# Autodesk Inventor assembly: Assembly
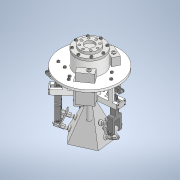
[picture p0: Inventor's stored thumbnail of the model, 180x180]
Saved by Autodesk Inventor 2021 (Build 250183000, 183)
## iProperties
Created: 2020-11-29
Part Number: Assembly
Document SubType Name: Assembly
Designer: awitc
Author: awitc
## Documents named in this file (36)
- C:\Users\awitc\Documents\Mechatronic Engineering\III rok\IndustrialRobots\GripperProject\Assembly.iam
- C:\Users\awitc\Documents\Mechatronic Engineering\III rok\IndustrialRobots\GripperProject\cup.ipt
- C:\Users\awitc\Documents\Mechatronic Engineering\III rok\IndustrialRobots\GripperProject\link.ipt
- C:\Users\awitc\Documents\Mechatronic Engineering\III rok\IndustrialRobots\GripperProject\finger.ipt
- C:\Users\awitc\Documents\Mechatronic Engineering\III rok\IndustrialRobots\GripperProject\actuatorLink.ipt
- C:\Users\awitc\Documents\Mechatronic Engineering\III rok\IndustrialRobots\GripperProject\bracket.ipt
- C:\Users\awitc\Documents\Mechatronic Engineering\III rok\IndustrialRobots\GripperProject\linkToActuator2.ipt
- C:\Users\awitc\Documents\Mechatronic Engineering\III rok\IndustrialRobots\GripperProject\linkToActuator3.ipt
- C:\Users\awitc\Documents\Mechatronic Engineering\III rok\IndustrialRobots\GripperProject\linkToActuator5.ipt
- C:\Users\awitc\Documents\Mechatronic Engineering\III rok\IndustrialRobots\GripperProject\linkToActuator4.ipt
- C:\Users\awitc\Documents\Mechatronic Engineering\III rok\IndustrialRobots\GripperProject\joint.ipt
- C:\Users\awitc\Documents\Mechatronic Engineering\III rok\IndustrialRobots\GripperProject\pneumaticActuator.ipt
- C:\Users\awitc\Documents\Mechatronic Engineering\III rok\IndustrialRobots\GripperProject\actuatorMountingPlate.ipt
- C:\Users\awitc\Documents\Mechatronic Engineering\III rok\IndustrialRobots\GripperProject\spacer.ipt
- C:\Users\awitc\Documents\Mechatronic Engineering\III rok\IndustrialRobots\GripperProject\vacuumGenerator.ipt
- C:\Users\awitc\Documents\Mechatronic Engineering\III rok\IndustrialRobots\GripperProject\mountingPlate.ipt
- C:\Users\awitc\Documents\Mechatronic Engineering\III rok\IndustrialRobots\GripperProject\pipeJoint.ipt
- C:\Users\awitc\Documents\Mechatronic Engineering\III rok\IndustrialRobots\GripperProject\customPin.ipt
- C:\Users\awitc\Documents\Inventor\Content Center Files\R2021\en-US\DIN 84\DIN 84 - M3 x 8.ipt
- C:\Users\awitc\Documents\Inventor\Content Center Files\R2021\en-US\DIN 84\DIN 84 - M1 x 8.ipt
- C:\Users\awitc\Documents\Inventor\Content Center Files\R2021\en-US\DIN 84\DIN 84 - M3 x 28.ipt
- C:\Users\awitc\Documents\Inventor\Content Center Files\R2021\en-US\DIN 439-2\DIN 439 - M3 x 0,5.ipt
- C:\Users\awitc\Documents\Inventor\Content Center Files\R2021\en-US\DIN 84\DIN 84 - M3 x 6.ipt
- C:\Users\awitc\Documents\Inventor\Content Center Files\R2021\en-US\DIN 125-1  A\DIN 125 - A 3,2.ipt
- C:\Users\awitc\Documents\Inventor\Content Center Files\R2021\en-US\DIN 84\DIN 84 - M3 x 14.ipt
- C:\Users\awitc\Documents\Mechatronic Engineering\III rok\IndustrialRobots\GripperProject\holder.ipt
- C:\Users\awitc\Documents\Inventor\Content Center Files\R2021\en-US\DIN 84\DIN 84 - M3 x 12.ipt
- C:\Users\awitc\Documents\Inventor\Content Center Files\R2021\en-US\DIN 84\DIN 84 - M3 x 25.ipt
- C:\Users\awitc\Documents\Mechatronic Engineering\III rok\IndustrialRobots\GripperProject\upperBasePart1.ipt
- C:\Users\awitc\Documents\Mechatronic Engineering\III rok\IndustrialRobots\GripperProject\upperBasePart2.ipt
- C:\Users\awitc\Documents\Mechatronic Engineering\III rok\IndustrialRobots\GripperProject\basePart1.ipt
- C:\Users\awitc\Documents\Mechatronic Engineering\III rok\IndustrialRobots\GripperProject\basePart2.ipt
- C:\Users\awitc\Documents\Mechatronic Engineering\III rok\IndustrialRobots\GripperProject\WK330.ipt
- C:\Users\awitc\Documents\Mechatronic Engineering\III rok\IndustrialRobots\GripperProject\sensorMount.ipt
- C:\Users\awitc\Documents\Mechatronic Engineering\III rok\IndustrialRobots\GripperProject\largePart.ipt
- C:\Users\awitc\Documents\Mechatronic Engineering\III rok\IndustrialRobots\GripperProject\Part4.ipt
## Components (142 placed, 35 different names)
1. bracket:1 — Insert:297, Insert:298, Insert:299, Insert:300, Insert:391, Insert:392
2. bracket:2 — Insert:301, Insert:302, Insert:303, Insert:304, Insert:395, Insert:396
3. bracket:3 — Insert:305, Insert:306, Insert:307, Insert:308, Insert:393, Insert:394
4. link:7 — Insert:144, Insert:145, Insert:169, Insert:174, Rigid:1, Insert:411, Insert:412, Mate:61, Flush:14
5. cup:14 — Insert:144
6. cup:16 — Insert:145, Insert:412
7. joint:1 — Insert:175, Rigid:1
8. pneumaticActuator:1 — Insert:159, Insert:160, Cylindrical:1
9. actuatorMountingPlate:1 — Insert:159, Insert:160, Insert:163, Insert:164, Insert:390, Flush:8
10. spacer:1 — Insert:163, Insert:164, Mate:59, Insert:410
11. vacuumGenerator:2 — Mate:36, Mate:37, Flush:1
12. mountingPlate:1 — Insert:339, Insert:340, Insert:341, Insert:342, Insert:343, Insert:344, Insert:345, Insert:346, Mate:58, Insert:409
13. pipeJoint:1 — Insert:169
14. pipeJoint:6 — Insert:174, Insert:411
15. finger:1 — Insert:175, Insert:255, Insert:294, Insert:311, Insert:312, Insert:324, Flush:9
16. link:8 — Insert:413, Insert:414
17. cup:17
18. cup:18 — Insert:413
19. joint:2 — Insert:189
20. pipeJoint:7
21. pipeJoint:8 — Insert:414
22. finger:2 — Insert:189, Insert:243, Insert:295, Insert:310, Insert:313, Insert:325, Flush:11
23. link:9 — Insert:415, Insert:416
24. cup:19
25. cup:20 — Insert:415
26. joint:3
27. pipeJoint:9
28. pipeJoint:10 — Insert:416
29. finger:3 — Insert:266, Insert:296, Insert:309, Insert:314, Insert:323, Flush:10
30. linkToActuator2:1 — Insert:244, Insert:245, Insert:292, Insert:293, Insert:397
31. linkToActuator3:1 — Insert:246, Insert:247, Insert:286, Insert:291, Insert:398
32. linkToActuator4:1 — Insert:245, Insert:246
33. linkToActuator5:1 — Insert:243, Insert:244
34. actuatorLink:1 — Insert:273, Cylindrical:1, Insert:274, Insert:275, Insert:315, Insert:316, Insert:317, Insert:318, Insert:319, Insert:320
35. linkToActuator5:2 — Insert:247, Insert:275
36. linkToActuator2:2 — Insert:288, Insert:289, Insert:401
37. linkToActuator3:2 — Insert:287, Insert:290, Insert:402
38. linkToActuator4:2
39. linkToActuator5:3 — Insert:255
40. linkToActuator5:4 — Insert:273
41. linkToActuator2:3 — Insert:265, Insert:282, Insert:284, Insert:399
42. linkToActuator3:3 — Insert:283, Insert:285, Insert:400
43. linkToActuator4:3
44. linkToActuator5:6 — Insert:274
45. linkToActuator5:7 — Insert:265, Insert:266
46. customPin:1 — Insert:282
47. customPin:2 — Insert:283
48. customPin:3 — Insert:285
49. customPin:4 — Insert:287
50. customPin:5 — Insert:286
51. customPin:6 — Insert:284
52. customPin:7 — Insert:288
53. customPin:8 — Insert:289
54. customPin:9 — Insert:290
55. customPin:10 — Insert:291
56. customPin:11 — Insert:292
57. customPin:12 — Insert:293
58. DIN 84 - replaced by DIN EN ISO 1207 M1 x 8:1 — Insert:299
59. DIN 84 - replaced by DIN EN ISO 1207 M1 x 8:2 — Insert:298
60. DIN 84 - replaced by DIN EN ISO 1207 M1 x 8:3 — Insert:297
61. DIN 84 - replaced by DIN EN ISO 1207 M1 x 8:4 — Insert:300
62. DIN 84 - replaced by DIN EN ISO 1207 M3 x 28:1 — Insert:296
63. DIN 84 - replaced by DIN EN ISO 1207 M3 x 28:2 — Insert:295
64. DIN 84 - replaced by DIN EN ISO 1207 M3 x 28:3 — Insert:294
65. DIN 84 - replaced by DIN EN ISO 1207 M1 x 8:5 — Insert:302
66. DIN 84 - replaced by DIN EN ISO 1207 M1 x 8:6 — Insert:303
67. DIN 84 - replaced by DIN EN ISO 1207 M1 x 8:7 — Insert:304
68. DIN 84 - replaced by DIN EN ISO 1207 M1 x 8:8 — Insert:301
69. DIN 84 - replaced by DIN EN ISO 1207 M1 x 8:10 — Insert:305
70. DIN 84 - replaced by DIN EN ISO 1207 M1 x 8:9 — Insert:308
71. DIN 84 - replaced by DIN EN ISO 1207 M1 x 8:11 — Insert:307
72. DIN 84 - replaced by DIN EN ISO 1207 M1 x 8:12 — Insert:306
73. DIN 439-2 - replaced by DIN EN 24035/28675 M3:1 — Insert:312
74. DIN 439-2 - replaced by DIN EN 24035/28675 M3:2 — Insert:314
75. DIN 439-2 - replaced by DIN EN 24035/28675 M3:4 — Insert:313
76. DIN 84 - replaced by DIN EN ISO 1207 M3 x 6:1 — Insert:309
77. DIN 84 - replaced by DIN EN ISO 1207 M3 x 6:2 — Insert:310
78. DIN 84 - replaced by DIN EN ISO 1207 M3 x 6:4 — Insert:311
79. DIN 84 - replaced by DIN EN ISO 1207 M3 x 6:5 — Insert:315
80. DIN 439-2 - replaced by DIN EN 24035/28675 M3:5 — Insert:316
81. DIN 439-2 - replaced by DIN EN 24035/28675 M3:6 — Insert:318
82. DIN 84 - replaced by DIN EN ISO 1207 M3 x 6:6 — Insert:317
83. DIN 84 - replaced by DIN EN ISO 1207 M3 x 6:7 — Insert:319
84. DIN 439-2 - replaced by DIN EN 24035/28675 M3:7 — Insert:320
85. DIN 125-1 A A 3,2:1 — Insert:323, Insert:330
86. DIN 125-1 A A 3,2:2 — Insert:336, Insert:407
87. DIN 125-1 A A 3,2:3 — Insert:337, Insert:406
88. DIN 125-1 A A 3,2:4 — Insert:324, Insert:331
89. DIN 125-1 A A 3,2:5 — Insert:325, Insert:332
90. DIN 125-1 A A 3,2:6 — Insert:333, Insert:405
91. DIN 125-1 A A 3,2:7 — Insert:338, Insert:408
92. DIN 125-1 A A 3,2:8 — Insert:334, Insert:404
93. DIN 125-1 A A 3,2:9 — Insert:335, Insert:403
94. DIN 439-2 - replaced by DIN EN 24035/28675 M3:8 — Insert:330
95. DIN 439-2 - replaced by DIN EN 24035/28675 M3:9 — Insert:331
96. DIN 439-2 - replaced by DIN EN 24035/28675 M3:10 — Insert:332
97. DIN 439-2 - replaced by DIN EN 24035/28675 M3:11 — Insert:333
98. DIN 439-2 - replaced by DIN EN 24035/28675 M3:12 — Insert:334
99. DIN 439-2 - replaced by DIN EN 24035/28675 M3:13 — Insert:335
100. DIN 439-2 - replaced by DIN EN 24035/28675 M3:14 — Insert:336
101. DIN 439-2 - replaced by DIN EN 24035/28675 M3:15 — Insert:337
102. DIN 439-2 - replaced by DIN EN 24035/28675 M3:16 — Insert:338
103. DIN 84 - replaced by DIN EN ISO 1207 M3 x 14:1 — Insert:345
104. DIN 84 - replaced by DIN EN ISO 1207 M3 x 14:2 — Insert:344
105. DIN 84 - replaced by DIN EN ISO 1207 M3 x 14:3 — Insert:343
106. DIN 84 - replaced by DIN EN ISO 1207 M3 x 14:4 — Insert:342
107. DIN 84 - replaced by DIN EN ISO 1207 M3 x 14:5 — Insert:341
108. DIN 84 - replaced by DIN EN ISO 1207 M3 x 14:6 — Insert:339
109. DIN 84 - replaced by DIN EN ISO 1207 M3 x 14:7 — Insert:340
110. DIN 84 - replaced by DIN EN ISO 1207 M3 x 14:9 — Insert:346
111. holder:1 — Mate:36, Mate:37, Flush:1, Insert:365, Insert:366, Insert:378, Insert:379
112. DIN 439-2 - replaced by DIN EN 24035/28675 M3:18 — Insert:365
113. DIN 439-2 - replaced by DIN EN 24035/28675 M3:19 — Insert:366
114. basePart1:1 — Mate:47, Flush:4, Mate:48, Mate:49, Flush:5, Mate:50, Mate:51, Flush:6, Insert:390, Mate:57, Flush:8
115. basePart2:1 — Mate:50, Mate:51, Flush:6, Insert:393, Insert:394, Insert:399, Insert:400, Flush:10, Insert:405, Insert:408
116. basePart2:2 — Mate:47, Flush:4, Mate:57, Insert:391, Insert:392, Insert:401, Insert:402, Flush:9, Insert:406, Insert:407
117. basePart2:3 — Mate:48, Mate:49, Flush:5, Insert:395, Insert:396, Insert:397, Insert:398, Flush:11, Insert:403, Insert:404
118. DIN 84 - replaced by DIN EN ISO 1207 M3 x 12:4 — Insert:381
119. DIN 84 - replaced by DIN EN ISO 1207 M3 x 12:5 — Insert:380
120. DIN 84 - replaced by DIN EN ISO 1207 M3 x 8:1 — Insert:389
121. upperBasePart2:1 — Mate:52, Mate:53, Mate:54, Mate:58, Insert:409
122. upperBasePart1:1 — Insert:369, Insert:370, Insert:371, Insert:372, Insert:373, Mate:52, Mate:53, Mate:54, Insert:376, Insert:377, Insert:378, Insert:379, Insert:380, Insert:381, Insert:382, Insert:383, Insert:384, Insert:385, Insert:386, Insert:387, Insert:388, Insert:389, Mate:59, Insert:410
123. DIN 84 - replaced by DIN EN ISO 1207 M3 x 25:2 — Insert:372
124. DIN 84 - replaced by DIN EN ISO 1207 M3 x 25:3 — Insert:373
125. DIN 84 - replaced by DIN EN ISO 1207 M3 x 25:5 — Insert:371
126. DIN 84 - replaced by DIN EN ISO 1207 M3 x 25:6 — Insert:369
127. DIN 84 - replaced by DIN EN ISO 1207 M3 x 25:7 — Insert:370
128. vacuumGenerator:3
129. holder:2 — Insert:376, Insert:377
130. DIN 439-2 - replaced by DIN EN 24035/28675 M3:20
131. DIN 439-2 - replaced by DIN EN 24035/28675 M3:21
132. DIN 84 - replaced by DIN EN ISO 1207 M3 x 12:6 — Insert:382
133. DIN 84 - replaced by DIN EN ISO 1207 M3 x 12:7 — Insert:383
134. DIN 84 - replaced by DIN EN ISO 1207 M3 x 8:2 — Insert:387
135. DIN 84 - replaced by DIN EN ISO 1207 M3 x 8:4 — Insert:385
136. DIN 84 - replaced by DIN EN ISO 1207 M3 x 8:5 — Insert:386
137. DIN 84 - replaced by DIN EN ISO 1207 M3 x 8:6 — Insert:388
138. DIN 84 - replaced by DIN EN ISO 1207 M3 x 8:7 — Insert:384
139. sensorMount:1 — Flush:12, Mate:60, Flush:13, Mate:61, Flush:14
140. WK330:1 — Flush:12, Mate:60, Flush:13
141. largePart:1 — Mate:62
142. Part4:1 — Mate:62
## Relationships (180: Insert 146, Mate 18, Flush 12, WeldJoint 3, CylindricalJoint 1)
- Insert:144: link:7 ↔ cup:14
- Insert:145: link:7 ↔ cup:16
- Insert:159: pneumaticActuator:1 ↔ actuatorMountingPlate:1
- Insert:160: pneumaticActuator:1 ↔ actuatorMountingPlate:1
- Insert:163: actuatorMountingPlate:1 ↔ spacer:1
- Insert:164: actuatorMountingPlate:1 ↔ spacer:1
- Insert:169: link:7 ↔ pipeJoint:1
- Insert:174: link:7 ↔ pipeJoint:6
- Insert:175: joint:1 ↔ finger:1
- Rigid:1 [WeldJoint]: link:7 ↔ joint:1
- [Insert]: link:8 ↔ cup:17
- [Insert]: link:8 ↔ cup:18
- [Insert]: link:8 ↔ pipeJoint:7
- [Insert]: link:8 ↔ pipeJoint:8
- [WeldJoint]: link:8 ↔ joint:2
- [Insert]: link:9 ↔ cup:19
- [Insert]: link:9 ↔ cup:20
- [Insert]: link:9 ↔ pipeJoint:9
- [Insert]: link:9 ↔ pipeJoint:10
- [Insert]: joint:3 ↔ finger:3
- [WeldJoint]: link:9 ↔ joint:3
- Insert:189: joint:2 ↔ finger:2
- Insert:243: finger:2 ↔ linkToActuator5:1
- Insert:244: linkToActuator2:1 ↔ linkToActuator5:1
- Insert:245: linkToActuator2:1 ↔ linkToActuator4:1
- Insert:246: linkToActuator3:1 ↔ linkToActuator4:1
- Insert:247: linkToActuator3:1 ↔ linkToActuator5:2
- [Insert]: linkToActuator2:2 ↔ linkToActuator5:3
- [Insert]: linkToActuator2:2 ↔ linkToActuator4:2
- [Insert]: linkToActuator3:2 ↔ linkToActuator4:2
- [Insert]: linkToActuator3:2 ↔ linkToActuator5:4
- Insert:255: finger:1 ↔ linkToActuator5:3
- [Insert]: linkToActuator2:3 ↔ linkToActuator4:3
- [Insert]: linkToActuator3:3 ↔ linkToActuator4:3
- [Insert]: linkToActuator3:3 ↔ linkToActuator5:6
- Insert:265: linkToActuator2:3 ↔ linkToActuator5:7
- Insert:266: finger:3 ↔ linkToActuator5:7
- Insert:273: actuatorLink:1 ↔ linkToActuator5:4
- Cylindrical:1: pneumaticActuator:1 ↔ actuatorLink:1
- Insert:274: actuatorLink:1 ↔ linkToActuator5:6
- Insert:275: actuatorLink:1 ↔ linkToActuator5:2
- Insert:282: linkToActuator2:3 ↔ customPin:1
- Insert:283: linkToActuator3:3 ↔ customPin:2
- Insert:284: linkToActuator2:3 ↔ customPin:6
- Insert:285: linkToActuator3:3 ↔ customPin:3
- Insert:286: linkToActuator3:1 ↔ customPin:5
- Insert:287: linkToActuator3:2 ↔ customPin:4
- Insert:288: linkToActuator2:2 ↔ customPin:7
- Insert:289: linkToActuator2:2 ↔ customPin:8
- Insert:290: linkToActuator3:2 ↔ customPin:9
- Insert:291: linkToActuator3:1 ↔ customPin:10
- Insert:292: linkToActuator2:1 ↔ customPin:11
- Insert:293: linkToActuator2:1 ↔ customPin:12
- Insert:294: finger:1 ↔ DIN 84 - replaced by DIN EN ISO 1207 M3 x 28:3
- Insert:295: finger:2 ↔ DIN 84 - replaced by DIN EN ISO 1207 M3 x 28:2
- Insert:296: finger:3 ↔ DIN 84 - replaced by DIN EN ISO 1207 M3 x 28:1
- Insert:297: bracket:1 ↔ DIN 84 - replaced by DIN EN ISO 1207 M1 x 8:3
- Insert:298: bracket:1 ↔ DIN 84 - replaced by DIN EN ISO 1207 M1 x 8:2
- Insert:299: bracket:1 ↔ DIN 84 - replaced by DIN EN ISO 1207 M1 x 8:1
- Insert:300: bracket:1 ↔ DIN 84 - replaced by DIN EN ISO 1207 M1 x 8:4
- Insert:301: bracket:2 ↔ DIN 84 - replaced by DIN EN ISO 1207 M1 x 8:8
- Insert:302: bracket:2 ↔ DIN 84 - replaced by DIN EN ISO 1207 M1 x 8:5
- Insert:303: bracket:2 ↔ DIN 84 - replaced by DIN EN ISO 1207 M1 x 8:6
- Insert:304: bracket:2 ↔ DIN 84 - replaced by DIN EN ISO 1207 M1 x 8:7
- Insert:305: bracket:3 ↔ DIN 84 - replaced by DIN EN ISO 1207 M1 x 8:10
- Insert:306: bracket:3 ↔ DIN 84 - replaced by DIN EN ISO 1207 M1 x 8:12
- Insert:307: bracket:3 ↔ DIN 84 - replaced by DIN EN ISO 1207 M1 x 8:11
- Insert:308: bracket:3 ↔ DIN 84 - replaced by DIN EN ISO 1207 M1 x 8:9
- Insert:309: finger:3 ↔ DIN 84 - replaced by DIN EN ISO 1207 M3 x 6:1
- Insert:310: finger:2 ↔ DIN 84 - replaced by DIN EN ISO 1207 M3 x 6:2
- Insert:311: finger:1 ↔ DIN 84 - replaced by DIN EN ISO 1207 M3 x 6:4
- Insert:312: finger:1 ↔ DIN 439-2 - replaced by DIN EN 24035/28675 M3:1
- Insert:313: finger:2 ↔ DIN 439-2 - replaced by DIN EN 24035/28675 M3:4
- Insert:314: finger:3 ↔ DIN 439-2 - replaced by DIN EN 24035/28675 M3:2
- Insert:315: actuatorLink:1 ↔ DIN 84 - replaced by DIN EN ISO 1207 M3 x 6:5
- Insert:316: actuatorLink:1 ↔ DIN 439-2 - replaced by DIN EN 24035/28675 M3:5
- Insert:317: actuatorLink:1 ↔ DIN 84 - replaced by DIN EN ISO 1207 M3 x 6:6
- Insert:318: actuatorLink:1 ↔ DIN 439-2 - replaced by DIN EN 24035/28675 M3:6
- Insert:319: actuatorLink:1 ↔ DIN 84 - replaced by DIN EN ISO 1207 M3 x 6:7
- Insert:320: actuatorLink:1 ↔ DIN 439-2 - replaced by DIN EN 24035/28675 M3:7
- Insert:323: finger:3 ↔ DIN 125-1 A A 3,2:1
- Insert:324: finger:1 ↔ DIN 125-1 A A 3,2:4
- Insert:325: finger:2 ↔ DIN 125-1 A A 3,2:5
- Insert:330: DIN 125-1 A A 3,2:1 ↔ DIN 439-2 - replaced by DIN EN 24035/28675 M3:8
- Insert:331: DIN 125-1 A A 3,2:4 ↔ DIN 439-2 - replaced by DIN EN 24035/28675 M3:9
- Insert:332: DIN 125-1 A A 3,2:5 ↔ DIN 439-2 - replaced by DIN EN 24035/28675 M3:10
- Insert:333: DIN 125-1 A A 3,2:6 ↔ DIN 439-2 - replaced by DIN EN 24035/28675 M3:11
- Insert:334: DIN 125-1 A A 3,2:8 ↔ DIN 439-2 - replaced by DIN EN 24035/28675 M3:12
- Insert:335: DIN 125-1 A A 3,2:9 ↔ DIN 439-2 - replaced by DIN EN 24035/28675 M3:13
- Insert:336: DIN 125-1 A A 3,2:2 ↔ DIN 439-2 - replaced by DIN EN 24035/28675 M3:14
- Insert:337: DIN 125-1 A A 3,2:3 ↔ DIN 439-2 - replaced by DIN EN 24035/28675 M3:15
- Insert:338: DIN 125-1 A A 3,2:7 ↔ DIN 439-2 - replaced by DIN EN 24035/28675 M3:16
- Insert:339: mountingPlate:1 ↔ DIN 84 - replaced by DIN EN ISO 1207 M3 x 14:6
- Insert:340: mountingPlate:1 ↔ DIN 84 - replaced by DIN EN ISO 1207 M3 x 14:7
- Insert:341: mountingPlate:1 ↔ DIN 84 - replaced by DIN EN ISO 1207 M3 x 14:5
- Insert:342: mountingPlate:1 ↔ DIN 84 - replaced by DIN EN ISO 1207 M3 x 14:4
- Insert:343: mountingPlate:1 ↔ DIN 84 - replaced by DIN EN ISO 1207 M3 x 14:3
- Insert:344: mountingPlate:1 ↔ DIN 84 - replaced by DIN EN ISO 1207 M3 x 14:2
- Insert:345: mountingPlate:1 ↔ DIN 84 - replaced by DIN EN ISO 1207 M3 x 14:1
- Insert:346: mountingPlate:1 ↔ DIN 84 - replaced by DIN EN ISO 1207 M3 x 14:9
- Mate:36: vacuumGenerator:2 ↔ holder:1
- Mate:37: vacuumGenerator:2 ↔ holder:1
- Flush:1: vacuumGenerator:2 ↔ holder:1
- Insert:365: holder:1 ↔ DIN 439-2 - replaced by DIN EN 24035/28675 M3:18
- Insert:366: holder:1 ↔ DIN 439-2 - replaced by DIN EN 24035/28675 M3:19
- Mate:47: basePart1:1 ↔ basePart2:2
- Flush:4: basePart1:1 ↔ basePart2:2
- Mate:48: basePart1:1 ↔ basePart2:3
- Mate:49: basePart1:1 ↔ basePart2:3
- Flush:5: basePart1:1 ↔ basePart2:3
- Mate:50: basePart1:1 ↔ basePart2:1
- Mate:51: basePart1:1 ↔ basePart2:1
- Flush:6: basePart1:1 ↔ basePart2:1
- Insert:369: upperBasePart1:1 ↔ DIN 84 - replaced by DIN EN ISO 1207 M3 x 25:6
- Insert:370: upperBasePart1:1 ↔ DIN 84 - replaced by DIN EN ISO 1207 M3 x 25:7
- Insert:371: upperBasePart1:1 ↔ DIN 84 - replaced by DIN EN ISO 1207 M3 x 25:5
- Insert:372: upperBasePart1:1 ↔ DIN 84 - replaced by DIN EN ISO 1207 M3 x 25:2
- Insert:373: upperBasePart1:1 ↔ DIN 84 - replaced by DIN EN ISO 1207 M3 x 25:3
- Mate:52: upperBasePart2:1 ↔ upperBasePart1:1
- Mate:53: upperBasePart2:1 ↔ upperBasePart1:1
- Mate:54: upperBasePart2:1 ↔ upperBasePart1:1
- [Mate]: vacuumGenerator:3 ↔ holder:2
- [Mate]: vacuumGenerator:3 ↔ holder:2
- [Flush]: vacuumGenerator:3 ↔ holder:2
- [Insert]: holder:2 ↔ DIN 439-2 - replaced by DIN EN 24035/28675 M3:20
- [Insert]: holder:2 ↔ DIN 439-2 - replaced by DIN EN 24035/28675 M3:21
- Insert:376: upperBasePart1:1 ↔ holder:2
- Insert:377: upperBasePart1:1 ↔ holder:2
- Insert:378: holder:1 ↔ upperBasePart1:1
- Insert:379: holder:1 ↔ upperBasePart1:1
- Insert:380: DIN 84 - replaced by DIN EN ISO 1207 M3 x 12:5 ↔ upperBasePart1:1
- Insert:381: DIN 84 - replaced by DIN EN ISO 1207 M3 x 12:4 ↔ upperBasePart1:1
- Insert:382: upperBasePart1:1 ↔ DIN 84 - replaced by DIN EN ISO 1207 M3 x 12:6
- Insert:383: upperBasePart1:1 ↔ DIN 84 - replaced by DIN EN ISO 1207 M3 x 12:7
- Insert:384: upperBasePart1:1 ↔ DIN 84 - replaced by DIN EN ISO 1207 M3 x 8:7
- Insert:385: upperBasePart1:1 ↔ DIN 84 - replaced by DIN EN ISO 1207 M3 x 8:4
- Insert:386: upperBasePart1:1 ↔ DIN 84 - replaced by DIN EN ISO 1207 M3 x 8:5
- Insert:387: upperBasePart1:1 ↔ DIN 84 - replaced by DIN EN ISO 1207 M3 x 8:2
- Insert:388: upperBasePart1:1 ↔ DIN 84 - replaced by DIN EN ISO 1207 M3 x 8:6
- Insert:389: DIN 84 - replaced by DIN EN ISO 1207 M3 x 8:1 ↔ upperBasePart1:1
- Insert:390: actuatorMountingPlate:1 ↔ basePart1:1
- Mate:57: basePart1:1 ↔ basePart2:2
- Flush:8: actuatorMountingPlate:1 ↔ basePart1:1
- Insert:391: bracket:1 ↔ basePart2:2
- Insert:392: bracket:1 ↔ basePart2:2
- Insert:393: bracket:3 ↔ basePart2:1
- Insert:394: bracket:3 ↔ basePart2:1
- Insert:395: bracket:2 ↔ basePart2:3
- Insert:396: bracket:2 ↔ basePart2:3
- Insert:397: linkToActuator2:1 ↔ basePart2:3
- Insert:398: linkToActuator3:1 ↔ basePart2:3
- Insert:399: linkToActuator2:3 ↔ basePart2:1
- Insert:400: linkToActuator3:3 ↔ basePart2:1
- Insert:401: linkToActuator2:2 ↔ basePart2:2
- Insert:402: linkToActuator3:2 ↔ basePart2:2
- Flush:9: finger:1 ↔ basePart2:2
- Flush:10: finger:3 ↔ basePart2:1
- Flush:11: finger:2 ↔ basePart2:3
- Mate:58: mountingPlate:1 ↔ upperBasePart2:1
- Insert:403: DIN 125-1 A A 3,2:9 ↔ basePart2:3
- Insert:404: DIN 125-1 A A 3,2:8 ↔ basePart2:3
- Insert:405: DIN 125-1 A A 3,2:6 ↔ basePart2:1
- Insert:406: DIN 125-1 A A 3,2:3 ↔ basePart2:2
- Insert:407: DIN 125-1 A A 3,2:2 ↔ basePart2:2
- Insert:408: DIN 125-1 A A 3,2:7 ↔ basePart2:1
- Mate:59: spacer:1 ↔ upperBasePart1:1
- Insert:409: mountingPlate:1 ↔ upperBasePart2:1
- Insert:410: spacer:1 ↔ upperBasePart1:1
- Insert:411: link:7 ↔ pipeJoint:6
- Insert:412: link:7 ↔ cup:16
- Insert:413: link:8 ↔ cup:18
- Insert:414: link:8 ↔ pipeJoint:8
- Insert:415: link:9 ↔ cup:20
- Insert:416: link:9 ↔ pipeJoint:10
- Flush:12: sensorMount:1 ↔ WK330:1
- Mate:60: sensorMount:1 ↔ WK330:1
- Flush:13: sensorMount:1 ↔ WK330:1
- Mate:61: link:7 ↔ sensorMount:1
- Flush:14: link:7 ↔ sensorMount:1
- Mate:62: largePart:1 ↔ Part4:1
## Named parameters: d365_d359 = 0 mm, d367_d364 = 0 mm, d368_d354 = 0 mm, d369_d287 = 0 mm, d370_d288 = 0 mm, d371_d359 = 0 mm, d372_d362 = 0 mm, d373_d364 = 0 mm, d374_d354 = 0 mm, d375_d287 = 0 mm, d376_d288 = 0 mm, d462_d455 = 0 mm, d463_d456 = 0 mm, d464_d457 = 0 mm, d465_d460 = 0 mm, d471_d456 = 0 mm, d472_d457 = 0 mm, d473_d460 = 0 mm, d635_d594 = 0 mm, d636_d595 = 0 mm, d637_d570 = 0 mm, d638_d571 = 0 mm, d639_d573 = 0 mm
